# Autodesk Inventor assembly: Right Structure
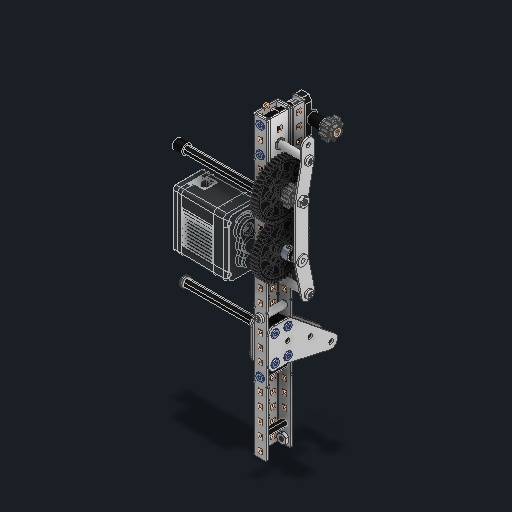
[picture p0: Inventor's stored thumbnail of the model, 512x512]
Saved by Autodesk Inventor 2025.1 (Build 291241000, 241)
## iProperties
Created: 2024-10-20
Part Number: Right Structure
Document SubType Name: Assembly
Designer: Averey Ku
Author: Averey Ku
## Documents named in this file (42)
- C:\Users\avere\VEX\High Stakes\CAD\V3\Tower\Right Structure\Right Structure.iam
- C:\Users\avere\VEX\High Stakes\CAD\V3\Tower\Right Structure\Right Alu C 1x2x1x23.ipt
- C:\Users\avere\VEX\High Stakes\CAD\ROBOPROS-CAD-Inventor\Structure\Standoff\Standoff .75.ipt
- C:\Users\avere\VEX\High Stakes\CAD\ROBOPROS-CAD-Inventor\Motion\Spacers\Washer Steel\SWasher .375 OD x .062500.ipt
- C:\Users\avere\VEX\High Stakes\CAD\ROBOPROS-CAD-Inventor\Structure\Hardware\Screw Steel - Star\SScrew Star Smooth .290.ipt
- C:\Users\avere\VEX\High Stakes\CAD\ROBOPROS-CAD-Inventor\Structure\Standoff\Standoff .875.ipt
- C:\Users\avere\VEX\High Stakes\CAD\ROBOPROS-CAD-Inventor\Structure\Hardware\Nut Nylon\Nut Nylon - White.ipt
- C:\Users\avere\VEX\High Stakes\CAD\V3\Tower\Right Structure\Right C Channel Coupler.ipt
- C:\Users\avere\VEX\High Stakes\CAD\ROBOPROS-CAD-Inventor\Structure\Hardware\Screw Shoulder Robosource\SScrew Shoulder Smooth .375 x .12.ipt
- C:\Users\avere\VEX\High Stakes\CAD\ROBOPROS-CAD-Inventor\Motion\Spacers\Spacer Nylon .375 OD\NSpacer .375 OD x .250.ipt
- C:\Users\avere\VEX\High Stakes\CAD\ROBOPROS-CAD-Inventor\Motion\Spacers\Spacer Nylon .375 OD\NSpacer .375 OD x .500.ipt
- C:\Users\avere\VEX\High Stakes\CAD\V3\Tower\Right Structure\Right Angle Brace Gusset.ipt
- C:\Users\avere\VEX\High Stakes\CAD\ROBOPROS-CAD-Inventor\Structure\Standoff\Standoff .50.ipt
- C:\Users\avere\VEX\High Stakes\CAD\ROBOPROS-CAD-Inventor\Structure\Hardware\Screw Shoulder Robosource\SScrew Shoulder Smooth .290 x .09.ipt
- C:\Users\avere\VEX\High Stakes\CAD\ROBOPROS-CAD-Inventor\Structure\Hardware\Screw Shoulder Robosource\SScrew Shoulder Smooth .500 x .04.ipt
- C:\Users\avere\VEX\High Stakes\CAD\ROBOPROS-CAD-Inventor\Structure\Standoff\Standoff 3.00.ipt
- C:\Users\avere\VEX\High Stakes\CAD\V3\Tower\Right Structure\Right 4-Post Standoff Retainer.ipt
- C:\Users\avere\VEX\High Stakes\CAD\ROBOPROS-CAD-Inventor\Structure\Hardware\Screw Steel - Star\SScrew Star Smooth .875.ipt
- C:\Users\avere\VEX\High Stakes\CAD\ROBOPROS-CAD-Inventor\Motion\Spacers\Spacer Nylon .375 OD\NSpacer .375 OD x .375.ipt
- C:\Users\avere\VEX\High Stakes\CAD\ROBOPROS-CAD-Inventor\Structure\Standoff.ipt
- C:\Users\avere\VEX\High Stakes\CAD\ROBOPROS-CAD-Inventor\Motion\Spacers\Washer Steel.ipt
- C:\Users\avere\VEX\High Stakes\CAD\ROBOPROS-CAD-Inventor\Structure\Hardware\Screw Steel - Star.ipt
- C:\Users\avere\VEX\High Stakes\CAD\ROBOPROS-CAD-Inventor\Structure\Hardware\Nut Nylon.ipt
- C:\Users\avere\VEX\High Stakes\CAD\ROBOPROS-CAD-Inventor\Structure\Hardware\Screw Shoulder Robosource.ipt
- C:\Users\avere\VEX\High Stakes\CAD\ROBOPROS-CAD-Inventor\Motion\Spacers\Spacer Nylon .375 OD.ipt
- C:\Users\avere\VEX\High Stakes\CAD\ROBOPROS-CAD-Inventor\Motion\Shaft HS\HS Pillow Bearing Block.ipt
- C:\Users\avere\VEX\High Stakes\CAD\ROBOPROS-CAD-Inventor\Structure\Angle\Aluminum 1x1\Alu Angle 1x1x3.ipt
- C:\Users\avere\VEX\High Stakes\CAD\ROBOPROS-CAD-Inventor\Motion\Spacers\Spacer Nylon .375 OD\NSpacer .375 OD x .125.ipt
- C:\Users\avere\VEX\High Stakes\CAD\ROBOPROS-CAD-Inventor\Motion\Shaft LS\Bearing Flat Low Profile.ipt
- C:\Users\avere\VEX\High Stakes\CAD\ROBOPROS-CAD-Inventor\Structure\Hardware\Screw Steel - Star\SScrew Star Smooth 1.750.ipt
- C:\Users\avere\VEX\High Stakes\CAD\ROBOPROS-CAD-Inventor\Structure\Nylon Standoff Rounded\Nylon Standoff .875.ipt
- C:\Users\avere\VEX\High Stakes\CAD\ROBOPROS-CAD-Inventor\Structure\Hardware\Screw Nylon - Pan Head\NScrew Pan Head Threaded .250.ipt
- C:\Users\avere\VEX\High Stakes\CAD\V3\Intake\Gearbox Right\Conveyer Gearbox Right.iam
- C:\Users\avere\VEX\High Stakes\CAD\ROBOPROS-CAD-Inventor\Motion\Spacers\Washer Steel\SWasher .375 OD x .015625.ipt
- C:\Users\avere\VEX\High Stakes\CAD\ROBOPROS-CAD-Inventor\Motion\Spacers\Washer Steel\SWasher .375 OD x .031250.ipt
- C:\Users\avere\VEX\High Stakes\CAD\ROBOPROS-CAD-Inventor\Structure\Hardware\Screw Steel - Star\SScrew Star Smooth 1.000.ipt
- C:\Users\avere\VEX\High Stakes\CAD\ROBOPROS-CAD-Inventor\Motion\Sprockets\6P Sprocket\6P 8T Sprocket, No Insert.iam
- C:\Users\avere\VEX\High Stakes\CAD\ROBOPROS-CAD-Inventor\Motion\Sprockets\6P Sprocket.iam
- C:\Users\avere\VEX\High Stakes\CAD\ROBOPROS-CAD-Inventor\Motion\Shaft HS\HS Spacer\HSpacer .5000.ipt
- C:\Users\avere\VEX\High Stakes\CAD\ROBOPROS-CAD-Inventor\Motion\Shaft HS\HS Spacer.ipt
- C:\Users\avere\VEX\High Stakes\CAD\ROBOPROS-CAD-Inventor\Electronics\Motors with Screws\SteelM-StarS.iam
- C:\Users\avere\VEX\High Stakes\CAD\ROBOPROS-CAD-Inventor\Electronics\Motors with Screws.iam
## Components (57 placed, 32 different names)
1. Right Alu C 1x2x1x23:1 — Mate:6, Insert:1, Insert:3, Insert:4, Insert:6, Insert:7, Insert:8, Mate:2, Insert:17, Mate:3, Insert:18, Mate:4, Insert:25, Insert:26, Mate:5, Insert:41, Mate:9, Insert:42, Insert:43, Insert:44, Insert:45, Insert:46, Insert:47, Insert:49, Insert:58, Mate:12
2. Standoff .75:1 — Insert:1, Insert:2
3. SWasher .375 OD x .062500:1 — Insert:2
4. SScrew Star Smooth .290:1 — Insert:6
5. Standoff .875:2 — Insert:3
6. Nut Nylon - White:1 — Insert:4
7. Right C Channel Coupler:1 — Insert:8, Mate:2, Insert:12, Insert:14, Mate:11
8. SScrew Shoulder Smooth .375 x .12:1 — Insert:7
9. NSpacer .375 OD x .250:1 — Insert:12, Insert:11
10. NSpacer .375 OD x .500:2 — Insert:11
11. NSpacer .375 OD x .250:3 — Insert:13
12. NSpacer .375 OD x .500:4 — Insert:14, Insert:13
13. Right Angle Brace Gusset:1 — Insert:17, Mate:3, Insert:19, Insert:20, Insert:22, Insert:21, Insert:24, Insert:30
14. Right Angle Brace Gusset:2 — Insert:18, Mate:4, Insert:23, Insert:31, Insert:59
15. NSpacer .375 OD x .500:5 — Insert:19
16. NSpacer .375 OD x .500:6 — Insert:20
17. Standoff .50:3 — Insert:22
18. NSpacer .375 OD x .500:7 — Insert:21
19. SScrew Shoulder Smooth .375 x .12:2 — Insert:23
20. SScrew Shoulder Smooth .290 x .09:3 — Insert:24
21. SScrew Shoulder Smooth .500 x .04:4 — Insert:25
22. Standoff 3.00:4 — Insert:29, Insert:32
23. Right 4-Post Standoff Retainer:1 — Insert:29, Insert:26, Mate:5
24. NSpacer .375 OD x .375:8 — Insert:32
25. HS Pillow Bearing Block:1 — Insert:56
26. Nut Nylon - White:8
27. Nut Nylon - White:9
28. Alu Angle 1x1x3:1
29. SWasher .375 OD x .062500:2 — Insert:41
30. NSpacer .375 OD x .125:9
31. NSpacer .375 OD x .125:10
32. Bearing Flat Low Profile:1
33. SWasher .375 OD x .062500:3 — Mate:9
34. SScrew Star Smooth 1.750:8 — Insert:43
35. SScrew Star Smooth 1.750:9 — Insert:42
36. Nylon Standoff .875:1 — Insert:44
37. Nylon Standoff .875:2 — Insert:45
38. NScrew Pan Head Threaded .250:1 — Insert:46
39. NScrew Pan Head Threaded .250:2 — Insert:47
40. Conveyer Gearbox Right:1 [sub-assembly] — Insert:49, Mate:11
41. SScrew Star Smooth 1.000:10 — Insert:50
42. NSpacer .375 OD x .250:11 — Insert:52, Insert:59
43. Standoff 3.00:5 — Insert:52, Insert:55
44. SWasher .375 OD x .015625:7 — Insert:54
45. SWasher .375 OD x .031250:8 — Insert:53, Insert:54
46. SWasher .375 OD x .062500:9 — Insert:53, Insert:55
47. 6P 8T Sprocket, No Insert:1 [sub-assembly] — Insert:57
48. HSpacer .5000:1 — Insert:56, Insert:57
49. SteelM-StarS:1 [sub-assembly] — Insert:58, Mate:12
50. Nut Nylon - White:4 — Insert:31
51. SScrew Star Smooth .875:4 — Insert:30, Insert:50
52. Nut Nylon - White:5
53. SScrew Star Smooth .875:5
54. Nut Nylon - White:6
55. SScrew Star Smooth .875:6
56. Nut Nylon - White:7
57. SScrew Star Smooth .875:7
## Component patterns: (4 elements, first: Nut Nylon - White:4 + SScrew Star Smooth .875:4)
## Relationships (60: Insert 50, Mate 10)
- Mate:6: Right Alu C 1x2x1x23:1
- Insert:1: Right Alu C 1x2x1x23:1 ↔ Standoff .75:1
- Insert:2: Standoff .75:1 ↔ SWasher .375 OD x .062500:1
- Insert:3: Right Alu C 1x2x1x23:1 ↔ Standoff .875:2
- Insert:4: Right Alu C 1x2x1x23:1 ↔ Nut Nylon - White:1
- Insert:6: Right Alu C 1x2x1x23:1 ↔ SScrew Star Smooth .290:1
- Insert:7: Right Alu C 1x2x1x23:1 ↔ SScrew Shoulder Smooth .375 x .12:1
- Insert:8: Right Alu C 1x2x1x23:1 ↔ Right C Channel Coupler:1
- Mate:2: Right Alu C 1x2x1x23:1 ↔ Right C Channel Coupler:1
- Insert:12: Right C Channel Coupler:1 ↔ NSpacer .375 OD x .250:1
- Insert:11: NSpacer .375 OD x .250:1 ↔ NSpacer .375 OD x .500:2
- Insert:14: Right C Channel Coupler:1 ↔ NSpacer .375 OD x .500:4
- Insert:13: NSpacer .375 OD x .250:3 ↔ NSpacer .375 OD x .500:4
- Insert:17 (12.7 mm): Right Alu C 1x2x1x23:1 ↔ Right Angle Brace Gusset:1
- Mate:3: Right Alu C 1x2x1x23:1 ↔ Right Angle Brace Gusset:1
- Insert:18: Right Alu C 1x2x1x23:1 ↔ Right Angle Brace Gusset:2
- Mate:4: Right Alu C 1x2x1x23:1 ↔ Right Angle Brace Gusset:2
- Insert:19: Right Angle Brace Gusset:1 ↔ NSpacer .375 OD x .500:5
- Insert:20: Right Angle Brace Gusset:1 ↔ NSpacer .375 OD x .500:6
- Insert:22: Right Angle Brace Gusset:1 ↔ Standoff .50:3
- Insert:21: Right Angle Brace Gusset:1 ↔ NSpacer .375 OD x .500:7
- Insert:23: Right Angle Brace Gusset:2 ↔ SScrew Shoulder Smooth .375 x .12:2
- Insert:24: Right Angle Brace Gusset:1 ↔ SScrew Shoulder Smooth .290 x .09:3
- Insert:25: Right Alu C 1x2x1x23:1 ↔ SScrew Shoulder Smooth .500 x .04:4
- Insert:29: Standoff 3.00:4 ↔ Right 4-Post Standoff Retainer:1
- Insert:26: Right Alu C 1x2x1x23:1 ↔ Right 4-Post Standoff Retainer:1
- Mate:5: Right Alu C 1x2x1x23:1 ↔ Right 4-Post Standoff Retainer:1
- Insert:31: Right Angle Brace Gusset:2 ↔ Nut Nylon - White:4
- Insert:30: Right Angle Brace Gusset:1 ↔ SScrew Star Smooth .875:4
- Insert:32: Standoff 3.00:4 ↔ NSpacer .375 OD x .375:8
- [Insert]: HS Pillow Bearing Block:1 ↔ Nut Nylon - White:9
- [Insert]: HS Pillow Bearing Block:1 ↔ Nut Nylon - White:8
- [Insert]: HS Pillow Bearing Block:1 ↔ Alu Angle 1x1x3:1
- [Mate]: HS Pillow Bearing Block:1 ↔ Alu Angle 1x1x3:1
- [Insert] (1.27 mm): NSpacer .375 OD x .125:10 ↔ Bearing Flat Low Profile:1
- [Insert] (1.27 mm): NSpacer .375 OD x .125:9 ↔ Bearing Flat Low Profile:1
- [Insert]: SWasher .375 OD x .062500:2 ↔ NSpacer .375 OD x .125:9
- [Insert]: NSpacer .375 OD x .125:10 ↔ SWasher .375 OD x .062500:3
- [Insert]: Alu Angle 1x1x3:1 ↔ Bearing Flat Low Profile:1
- [Mate]: Alu Angle 1x1x3:1 ↔ SWasher .375 OD x .062500:3
- Insert:41: Right Alu C 1x2x1x23:1 ↔ SWasher .375 OD x .062500:2
- Mate:9: Right Alu C 1x2x1x23:1 ↔ SWasher .375 OD x .062500:3
- Insert:42: Right Alu C 1x2x1x23:1 ↔ SScrew Star Smooth 1.750:9
- Insert:43: Right Alu C 1x2x1x23:1 ↔ SScrew Star Smooth 1.750:8
- Insert:44: Right Alu C 1x2x1x23:1 ↔ Nylon Standoff .875:1
- Insert:45: Right Alu C 1x2x1x23:1 ↔ Nylon Standoff .875:2
- Insert:46: Right Alu C 1x2x1x23:1 ↔ NScrew Pan Head Threaded .250:1
- Insert:47: Right Alu C 1x2x1x23:1 ↔ NScrew Pan Head Threaded .250:2
- Insert:49: Right Alu C 1x2x1x23:1 ↔ Conveyer Gearbox Right:1
- Mate:11: Right C Channel Coupler:1 ↔ Conveyer Gearbox Right:1
- Insert:50: SScrew Star Smooth 1.000:10 ↔ SScrew Star Smooth .875:4
- Insert:52: NSpacer .375 OD x .250:11 ↔ Standoff 3.00:5
- Insert:53: SWasher .375 OD x .031250:8 ↔ SWasher .375 OD x .062500:9
- Insert:54: SWasher .375 OD x .015625:7 ↔ SWasher .375 OD x .031250:8
- Insert:55: Standoff 3.00:5 ↔ SWasher .375 OD x .062500:9
- Insert:56: HS Pillow Bearing Block:1 ↔ HSpacer .5000:1
- Insert:57: 6P 8T Sprocket, No Insert:1 ↔ HSpacer .5000:1
- Insert:58: Right Alu C 1x2x1x23:1 ↔ SteelM-StarS:1
- Mate:12: Right Alu C 1x2x1x23:1 ↔ SteelM-StarS:1
- Insert:59: Right Angle Brace Gusset:2 ↔ NSpacer .375 OD x .250:11
## Named parameters: d42_d46 = 0 mm, d43_d47 = 0 mm, d44_d50 = 1.27 mm
